# Autodesk Inventor assembly: assembly2
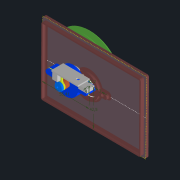
[picture p0: Inventor's stored thumbnail of the model, 180x180]
Saved by Autodesk Inventor 2021 (Build 250183000, 183)
## iProperties
Created: 2021-12-12
Part Number: assembly2
Document SubType Name: Assembly
Designer: Juan M. Casillas
Author: Juan M. Casillas
## Documents named in this file (10)
- K:\3DPrinting\3DModels\3party\ElectricEel_rueca\medidor\v1\assembly2.iam
- K:\3DPrinting\3DModels\3party\ElectricEel_rueca\medidor\v1\carrete.ipt
- K:\3DPrinting\3DModels\3party\ElectricEel_rueca\medidor\rodamiento.ipt
- K:\3DPrinting\3DModels\3party\ElectricEel_rueca\medidor\v1\separador_5mm.ipt
- K:\3DPrinting\3DModels\3party\ElectricEel_rueca\medidor\cierre.ipt
- K:\3DPrinting\3DModels\3party\ElectricEel_rueca\medidor\v1\encoder_selector.ipt
- K:\3DPrinting\3DModels\3party\ElectricEel_rueca\medidor\irencoder_footprint.ipt
- K:\3DPrinting\3DModels\3party\ElectricEel_rueca\medidor\v1\separador_10mm.ipt
- K:\3DPrinting\3DModels\3party\ElectricEel_rueca\medidor\v1\caja.ipt
- K:\3DPrinting\3DModels\3party\ElectricEel_rueca\medidor\v1\caja_down.ipt
## Components (9 placed, 9 different names)
1. carrete:1 — Mate:1
2. rodamiento:1 — Mate:2, Mate:3, Mate:5
3. separador_5mm:2 — Mate:1, Mate:2
4. cierre:1
5. encoder_selector:1 — Mate:4
6. irencoder_footprint:1
7. separador_10mm:1 — Mate:3, Mate:4, Mate:6
8. caja:1 — Mate:5
9. caja_down:1 — Mate:6
## Relationships (6: Mate 6)
- Mate:1: carrete:1 ↔ separador_5mm:2
- Mate:2: rodamiento:1 ↔ separador_5mm:2
- Mate:3: rodamiento:1 ↔ separador_10mm:1
- Mate:4: encoder_selector:1 ↔ separador_10mm:1
- Mate:5: rodamiento:1 ↔ caja:1
- Mate:6: separador_10mm:1 ↔ caja_down:1
